# Autodesk Inventor assembly: Motedius_Gelenkfuß_10_PA_M6x60
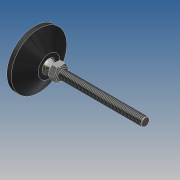
[picture p0: Inventor's stored thumbnail of the model, 180x180]
Saved by Autodesk Inventor 2015 (Build 190159000, 159)
## iProperties
Created: 2015-01-09
Part Number: Motedius_Gelenkfuß_10_PA_M6x60
Document SubType Name: Assembly
Designer: Marc
Author: Marc
## Documents named in this file (4)
- E:\Modellflieger\3D Drucker\MotediusQR 500mm\Motedius Gelenkfuß 10 PA\Motedius_Gelenkfuß_10_PA_M6x60.iam
- E:\Modellflieger\3D Drucker\MotediusQR 500mm\Motedius Gelenkfuß 10 PA\M6x60.ipt
- E:\Modellflieger\3D Drucker\MotediusQR 500mm\Motedius Gelenkfuß 10 PA\Plastikfuß_40mm.ipt
- C:\Users\Marc\Documents\Inventor\Content Center Files\R2015\de-DE\DIN 934\DIN 934 - M6 x 1.ipt
## Components (3 placed, 3 different names)
1. M6x60:1 — Einfügen:1, Einfügen:2
2. Plastikfuß_40mm:1 — Einfügen:1
3. DIN 934 - ersetzt durch DIN EN 24032/28673/28674 M6:1 — Einfügen:2
## Relationships (2: Insert 2)
- Einfügen:1 [Insert] (6.5 mm): M6x60:1 ↔ Plastikfuß_40mm:1
- Einfügen:2 [Insert] (2.6 mm): M6x60:1 ↔ DIN 934 - ersetzt durch DIN EN 24032/28673/28674 M6:1
